# Autodesk Inventor assembly: 000-A-000
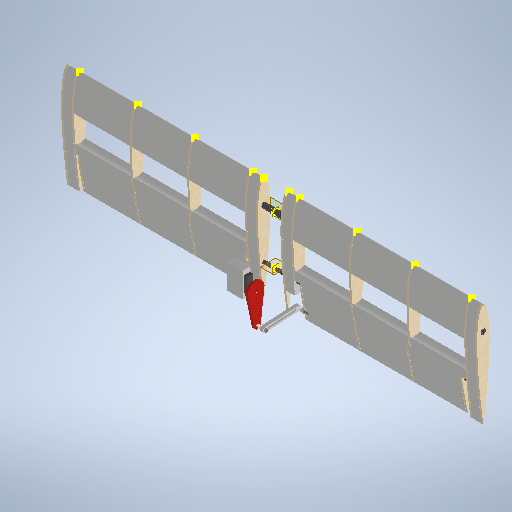
[picture p0: Inventor's stored thumbnail of the model, 512x512]
Saved by Autodesk Inventor 2025.2 (Build 292293000, 293)
## iProperties
Created: 2025-01-11
Part Number: 000-A-000
Document SubType Name: Assembly
Designer: lachl
Category: <PROJECT CATAGORY>
Title: <TITLE>
Author: lachl
Revision Number: A
## Documents named in this file (27)
- C:\Users\lachl\OneDrive - University of Bristol\Full assembly\HTP & Elevator\6A-002.iam
- C:\Users\lachl\OneDrive - University of Bristol\Full assembly\HTP & Elevator\6P-001.ipt
- C:\Users\lachl\OneDrive - University of Bristol\Full assembly\HTP & Elevator\6P-002.ipt
- C:\Users\lachl\OneDrive - University of Bristol\Full assembly\HTP & Elevator\6P-003.ipt
- C:\Users\lachl\OneDrive - University of Bristol\Full assembly\HTP & Elevator\6P-004.ipt
- C:\Users\lachl\OneDrive - University of Bristol\Full assembly\HTP & Elevator\6P-005.ipt
- C:\Users\lachl\OneDrive - University of Bristol\Full assembly\HTP & Elevator\6P-006.ipt
- C:\Users\lachl\OneDrive - University of Bristol\Full assembly\HTP & Elevator\6P-007.ipt
- C:\Users\lachl\OneDrive - University of Bristol\Full assembly\HTP & Elevator\6P-008.ipt
- C:\Users\lachl\OneDrive - University of Bristol\Full assembly\HTP & Elevator\6P-009.ipt
- C:\Users\lachl\OneDrive - University of Bristol\Full assembly\HTP & Elevator\6P-010.ipt
- C:\Users\lachl\OneDrive - University of Bristol\Full assembly\HTP & Elevator\6P-011.ipt
- C:\Users\lachl\OneDrive - University of Bristol\Full assembly\HTP & Elevator\6P-013.ipt
- C:\Users\lachl\OneDrive - University of Bristol\Full assembly\HTP & Elevator\6P-012.ipt
- C:\Users\lachl\OneDrive - University of Bristol\Full assembly\HTP & Elevator\6P-015.ipt
- C:\Users\lachl\OneDrive - University of Bristol\Full assembly\HTP & Elevator\Foam next to elevator.ipt
- C:\Users\lachl\OneDrive - University of Bristol\Full assembly\HTP & Elevator\Foam sandwich next to mechanism.ipt
- C:\Users\lachl\Documents\Inventor\Content Center Files\R2025\en-US\GB_T 5782-2000\Bolt GB_T 5782 M2.5 x 20.ipt
- C:\Users\lachl\OneDrive - University of Bristol\Full assembly\HTP & Elevator\spacer 3.5mm.ipt
- C:\Users\lachl\Documents\Inventor\Content Center Files\R2025\en-US\AS 1112 (2)\AS 1112 - M2.5  Type 5.ipt
- C:\Users\lachl\OneDrive - University of Bristol\Full assembly\HTP & Elevator\6P-016.ipt
- C:\Users\lachl\OneDrive - University of Bristol\Full assembly\HTP & Elevator\6P-017.ipt
- C:\Users\lachl\OneDrive - University of Bristol\Full assembly\HTP & Elevator\Servo mount top v2.ipt
- C:\Users\lachl\OneDrive - University of Bristol\Full assembly\HTP & Elevator\elevator next to mechanism.ipt
- C:\Users\lachl\OneDrive - University of Bristol\Full assembly\HTP & Elevator\6P-016 cutout.ipt
- C:\Users\lachl\OneDrive - University of Bristol\Full assembly\HTP & Elevator\spacer 4.5mm.ipt
- C:\Users\me19654\OneDrive - University of Bristol\PhD Project\005 Design (CAD and schematics)\001 Wind Tunnel\CAD Library\001-A-017 CONTRACTION ASSY.iam
## Components (59 placed, 25 different names)
1. 6P-001:1 — Rotational:122, Rotational:124
2. 6P-002:1 — Rigid:108, Cylindrical:116, Rotational:138
3. 6P-003:1 — Rotational:124
4. 6P-003:2 — Rotational:114, Rotational:122
5. 6P-003:3
6. 6P-004:2
7. 6P-003:4
8. 6P-003:5
9. 6P-005:1
10. 6P-005:2
11. 6P-005:3
12. 6P-005:4
13. 6P-005:5
14. 6P-005:6
15. 6P-006:1 — Rigid:112
16. 6P-006:2 — Rigid:116, Rigid:117
17. 6P-006:3 — Rigid:115
18. 6P-006:4 — Rigid:113, Rigid:114
19. 6P-007:1
20. 6P-007:2
21. 6P-008:1
22. 6P-009:1
23. 6P-010:1
24. 6P-010:2 — Rigid:126, Rigid:127
25. 6P-010:3
26. 6P-010:4
27. 6P-010:5 — Rigid:125
28. 6P-010:6
29. 6P-010:7 — Rigid:128, Rigid:129
30. 6P-011:1 — Rotational:133, Cylindrical:119, Rigid:130, Rotational:138
31. 6P-013:1 — Rigid:108
32. 6P-013:2
33. 6P-013:3
34. 6P-006:5 — Rotational:126, Rotational:127
35. 6P-012:1
36. 6P-012:2
37. 6P-015:1 — Rotational:139
38. Foam next to elevator:1 — Rigid:117
39. Foam next to elevator:2 — Rigid:112
40. Foam next to elevator:3 — Rigid:116
41. Foam next to elevator:4 — Rigid:114
42. Foam next to elevator:5 — Rigid:113
43. Foam next to elevator:6 — Rigid:115
44. Foam sandwich next to mechanism:1 — Rotational:114, Cylindrical:116, Rotational:126, Rotational:127
45. Bolt GB/T 5782-2000 M2.5x20:1 — Rotational:135, Cylindrical:119
46. Bolt GB/T 5782-2000 M2.5x20:2 — Cylindrical:118, Rotational:141
47. spacer 3.5mm:2 — Rotational:142, Rotational:143
48. AS 1112 (2) - Metric M2.5  Type 5:1 — Rotational:137
49. AS 1112 (2) - Metric M2.5  Type 5:2 — Rotational:133
50. 6P-016:1 — Rotational:140, Rotational:141, Rotational:142
51. 6P-017:1 — Rotational:135, Cylindrical:118, Rotational:137, Rotational:144, Rotational:145
52. Servo mount top v2:1 — Rigid:124
53. Servo mount top v2:2 — Rigid:124
54. elevator next to mechanism:1 — Rigid:125, Rigid:126
55. elevator next to mechanism:2 — Rigid:127, Rigid:128
56. elevator next to mechanism:3 — Rigid:129, Rigid:130
57. 6P-016 cutout:1 — Rotational:139, Rotational:140
58. spacer 3.5mm:4 — Rotational:143, Rotational:144
59. spacer 4.5mm:1 — Rotational:145
## Relationships (61: WeldJoint 40, RevoluteJoint 16, CylindricalJoint 4, Mate 1)
- [WeldJoint]: 6P-003:1 ↔ 6P-004:2
- [WeldJoint]: 6P-003:3 ↔ 6P-004:2
- [CylindricalJoint]: 6P-002:1 ↔ 6P-004:2
- [WeldJoint]: 6P-003:3 ↔ 6P-005:1
- [WeldJoint]: 6P-005:1 ↔ 6P-006:2
- [WeldJoint]: 6P-005:3 ↔ 6P-006:2
- [WeldJoint]: 6P-005:3 ↔ 6P-006:1
- [WeldJoint]: 6P-005:4 ↔ 6P-006:1
- [WeldJoint]: 6P-003:4 ↔ 6P-005:4
- [WeldJoint]: 6P-005:2 ↔ 6P-006:3
- [WeldJoint]: 6P-005:5 ↔ 6P-006:3
- [WeldJoint]: 6P-005:5 ↔ 6P-006:4
- [WeldJoint]: 6P-005:6 ↔ 6P-006:4
- [WeldJoint]: 6P-003:5 ↔ 6P-005:6
- [WeldJoint]: 6P-003:4 ↔ 6P-009:1
- [WeldJoint]: 6P-007:1 ↔ 6P-009:1
- [WeldJoint]: 6P-003:5 ↔ 6P-008:1
- [WeldJoint]: 6P-007:2 ↔ 6P-008:1
- [WeldJoint]: 6P-010:4 ↔ 6P-013:1
- [WeldJoint]: 6P-010:3 ↔ 6P-013:1
- [WeldJoint]: 6P-010:3 ↔ 6P-013:3
- [WeldJoint]: 6P-010:6 ↔ 6P-013:3
- [WeldJoint]: 6P-010:6 ↔ 6P-013:2
- [WeldJoint]: 6P-010:1 ↔ 6P-013:2
- [WeldJoint]: 6P-005:2 ↔ 6P-006:5
- [Mate]: 6P-001:1 ↔ 6P-002:1
- [WeldJoint]: 6P-002:1 ↔ 6P-012:1
- [WeldJoint]: 6P-002:1 ↔ 6P-012:2
- Rigid:108 [WeldJoint] (-41.5 mm): 6P-002:1 ↔ 6P-013:1
- Rigid:112 [WeldJoint]: 6P-006:1 ↔ Foam next to elevator:2
- Rigid:113 [WeldJoint]: 6P-006:4 ↔ Foam next to elevator:5
- Rigid:114 [WeldJoint]: 6P-006:4 ↔ Foam next to elevator:4
- Rigid:115 [WeldJoint]: 6P-006:3 ↔ Foam next to elevator:6
- Rigid:116 [WeldJoint]: 6P-006:2 ↔ Foam next to elevator:3
- Rigid:117 [WeldJoint]: 6P-006:2 ↔ Foam next to elevator:1
- Rotational:114 [RevoluteJoint]: 6P-003:2 ↔ Foam sandwich next to mechanism:1
- Cylindrical:116: 6P-002:1 ↔ Foam sandwich next to mechanism:1
- Rotational:122 [RevoluteJoint] (17.5 mm): 6P-001:1 ↔ 6P-003:2
- Rotational:124 [RevoluteJoint] (-17.5 mm): 6P-001:1 ↔ 6P-003:1
- Rotational:126 [RevoluteJoint]: 6P-006:5 ↔ Foam sandwich next to mechanism:1
- Rotational:127 [RevoluteJoint]: 6P-006:5 ↔ Foam sandwich next to mechanism:1
- Rotational:133 [RevoluteJoint]: 6P-011:1 ↔ AS 1112 (2) - Metric M2.5  Type 5:2
- Rotational:135 [RevoluteJoint]: Bolt GB/T 5782-2000 M2.5x20:1 ↔ 6P-017:1
- Cylindrical:118: Bolt GB/T 5782-2000 M2.5x20:2 ↔ 6P-017:1
- Cylindrical:119: 6P-011:1 ↔ Bolt GB/T 5782-2000 M2.5x20:1
- Rotational:137 [RevoluteJoint]: AS 1112 (2) - Metric M2.5  Type 5:1 ↔ 6P-017:1
- Rigid:124 [WeldJoint]: Servo mount top v2:1 ↔ Servo mount top v2:2
- Rigid:125 [WeldJoint]: 6P-010:5 ↔ elevator next to mechanism:1
- Rigid:126 [WeldJoint]: 6P-010:2 ↔ elevator next to mechanism:1
- Rigid:127 [WeldJoint]: 6P-010:2 ↔ elevator next to mechanism:2
- Rigid:128 [WeldJoint]: 6P-010:7 ↔ elevator next to mechanism:2
- Rigid:129 [WeldJoint]: 6P-010:7 ↔ elevator next to mechanism:3
- Rigid:130 [WeldJoint]: 6P-011:1 ↔ elevator next to mechanism:3
- Rotational:138 [RevoluteJoint] (43.5 mm): 6P-002:1 ↔ 6P-011:1
- Rotational:139 [RevoluteJoint]: 6P-015:1 ↔ 6P-016 cutout:1
- Rotational:140 [RevoluteJoint]: 6P-016:1 ↔ 6P-016 cutout:1
- Rotational:141 [RevoluteJoint]: Bolt GB/T 5782-2000 M2.5x20:2 ↔ 6P-016:1
- Rotational:142 [RevoluteJoint]: spacer 3.5mm:2 ↔ 6P-016:1
- Rotational:143 [RevoluteJoint]: spacer 3.5mm:2 ↔ spacer 3.5mm:4
- Rotational:144 [RevoluteJoint]: 6P-017:1 ↔ spacer 3.5mm:4
- Rotational:145 [RevoluteJoint]: 6P-017:1 ↔ spacer 4.5mm:1
